# Autodesk Inventor assembly: CAD Model of Bridge Assembly
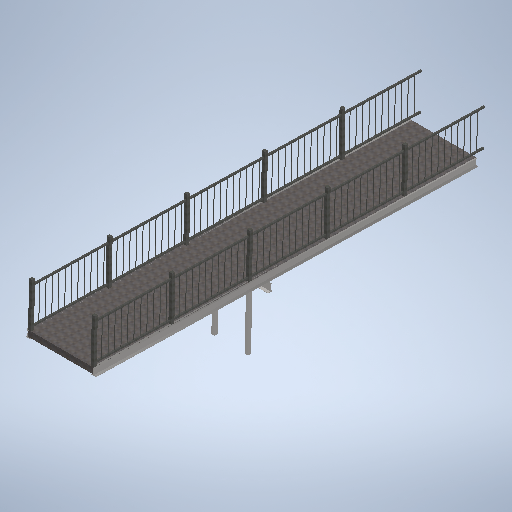
[picture p0: Inventor's stored thumbnail of the model, 512x512]
Saved by Autodesk Inventor 2025 (Build 290162000, 162)
## iProperties
Created: 2024-06-26
Part Number: CAD Model of Bridge Assembly
Document SubType Name: Assembly
Designer: track
Author: track
## Documents named in this file (7)
- C:\Users\track\OneDrive\Documents\USC-walking-bridges\Bridge_A\CAD_model\CAD Model of Bridge Assembly.iam
- C:\Users\track\OneDrive\Documents\USC-walking-bridges\Bridge_A\CAD_model\Concrete Walkway.ipt
- C:\Users\track\OneDrive\Documents\USC-walking-bridges\Bridge_A\CAD_model\Long I-Beam.ipt
- C:\Users\track\OneDrive\Documents\USC-walking-bridges\Bridge_A\CAD_model\Cylinder Supports.ipt
- C:\Users\track\OneDrive\Documents\USC-walking-bridges\Bridge_A\CAD_model\Short I-Beam.ipt
- C:\Users\track\OneDrive\Documents\USC-walking-bridges\Bridge_A\CAD_model\Railing.ipt
- C:\Users\track\OneDrive\Documents\USC-walking-bridges\Bridge_A\CAD_model\Cross Supports.ipt
## Components (16 placed, 6 different names)
1. Concrete Walkway:1 — Rigid:1, Rigid:2, Rigid:3, Mate:1, Mate:2, Flush:2
2. Long I-Beam:1 — Rigid:1, Mate:3, Flush:1, Mate:4
3. Long I-Beam:2 — Rigid:2
4. Cylinder Supports:1 — Mate:5, Mate:6
5. Short I-Beam:1 — Flush:1, Mate:4, Flush:2, Mate:5, Mate:6
6. Cross Supports:1 — Mate:1, Mate:2, Mate:3
7. Railing:1 — Rigid:3
8. Railing:2
9. Railing:3
10. Railing:4
11. Railing:5
12. Railing:6
13. Railing:7
14. Railing:8
15. Railing:9
16. Railing:10
## Component patterns: (10 elements, first: Railing:1)
## Relationships (11: Mate 6, WeldJoint 3, Flush 2)
- Rigid:1 [WeldJoint]: Concrete Walkway:1 ↔ Long I-Beam:1
- Rigid:2 [WeldJoint]: Concrete Walkway:1 ↔ Long I-Beam:2
- Rigid:3 [WeldJoint]: Concrete Walkway:1 ↔ Railing:1
- Mate:1 (381 mm): Concrete Walkway:1 ↔ Cross Supports:1
- Mate:2: Concrete Walkway:1 ↔ Cross Supports:1
- Mate:3: Long I-Beam:1 ↔ Cross Supports:1
- Flush:1 (-120.65 mm): Long I-Beam:1 ↔ Short I-Beam:1
- Mate:4: Long I-Beam:1 ↔ Short I-Beam:1
- Flush:2 (4375.15 mm): Concrete Walkway:1 ↔ Short I-Beam:1
- Mate:5: Cylinder Supports:1 ↔ Short I-Beam:1
- Mate:6 (-533.4 mm): Cylinder Supports:1 ↔ Short I-Beam:1
